# Autodesk Inventor assembly: oikon
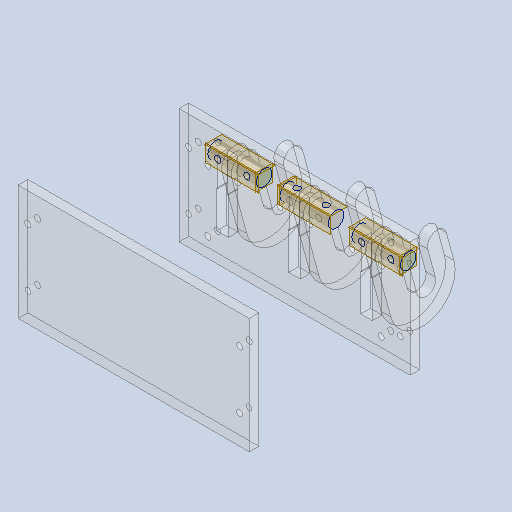
[picture p0: Inventor's stored thumbnail of the model, 512x512]
Saved by Autodesk Inventor 2025.2 (Build 292293000, 293)
## iProperties
Created: 2025-02-28
Part Number: oikon
Document SubType Name: Assembly
Designer: haruy
Author: haruy
## Documents named in this file (5)
- C:\Users\haruy\Documents\ロボコン\NHK2025\cad\nagahisa\oikon\oikon.iam
- C:\Users\haruy\Documents\ロボコン\NHK2025\cad\nagahisa\oikon\part1.ipt
- C:\Users\haruy\Documents\ロボコン\NHK2025\cad\nagahisa\oikon\part2.ipt
- C:\Users\haruy\Documents\ロボコン\NHK2025\cad\nagahisa\oikon\part3.ipt
- C:\Users\haruy\Documents\ロボコン\NHK2025\cad\nagahisa\oikon\part4.ipt
## Components (8 placed, 4 different names)
1. part1:1 — メイト:1, メイト:2, フラッシュ:1, メイト:3, フラッシュ:2, フラッシュ:3, フラッシュ:4, メイト:4
2. part2:1 — メイト:1, メイト:2, フラッシュ:2, メイト:5, 挿入:1
3. part2:2 — フラッシュ:4, メイト:4, メイト:5, 挿入:2
4. part2:3 — フラッシュ:1, メイト:3, フラッシュ:3, 挿入:3
5. part3:1 — 挿入:1
6. part3:2 — 挿入:2
7. part3:3 — 挿入:3
8. part4:1
## Relationships (12: Mate 5, Flush 4, Insert 3)
- メイト:1 [Mate] (-10 mm): part1:1 ↔ part2:1
- メイト:2 [Mate]: part1:1 ↔ part2:1
- フラッシュ:1 [Flush] (10 mm): part1:1 ↔ part2:3
- メイト:3 [Mate]: part1:1 ↔ part2:3
- フラッシュ:2 [Flush] (14 mm): part1:1 ↔ part2:1
- フラッシュ:3 [Flush] (14 mm): part1:1 ↔ part2:3
- フラッシュ:4 [Flush] (14 mm): part1:1 ↔ part2:2
- メイト:4 [Mate]: part1:1 ↔ part2:2
- メイト:5 [Mate] (12.2 mm): part2:1 ↔ part2:2
- 挿入:1 [Insert] (-10.1 mm): part2:1 ↔ part3:1
- 挿入:2 [Insert] (10.1 mm): part2:2 ↔ part3:2
- 挿入:3 [Insert] (10.1 mm): part2:3 ↔ part3:3
